# Autodesk Inventor assembly: Assembly3
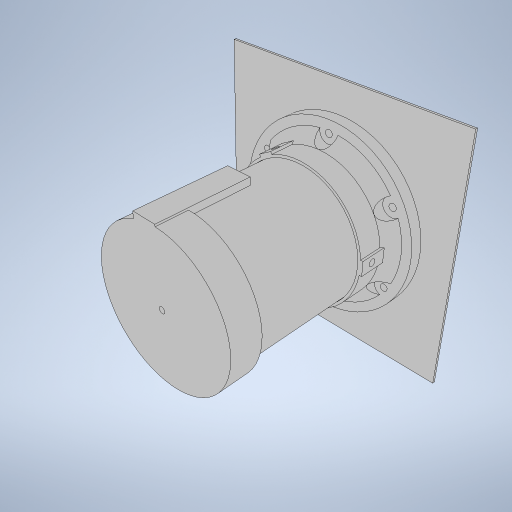
[picture p0: Inventor's stored thumbnail of the model, 512x512]
Saved by Autodesk Inventor 2023 (Build 270158000, 158)
## iProperties
Created: 2023-04-27
Part Number: Assembly3
Document SubType Name: Assembly
Designer: alexa
Author: alexa
## Documents named in this file (5)
- D:\Projects\Mushroom\Assembly3.iam
- D:\Projects\Mushroom\uppe sheet.ipt
- D:\Projects\Mushroom\holding ring.ipt
- D:\Projects\Mushroom\Pipe.ipt
- D:\Projects\Mushroom\Disc.ipt
## Components (4 placed, 4 different names)
1. uppe sheet:1 — Mate:1, Insert:1, Insert:2
2. holding ring:1 — Mate:1, Insert:1
3. Pipe:1 — Insert:2, Insert:3
4. Disc:1 — Insert:3
## Relationships (4: Insert 3, Mate 1)
- Mate:1: uppe sheet:1 ↔ holding ring:1
- Insert:1: uppe sheet:1 ↔ holding ring:1
- Insert:2: uppe sheet:1 ↔ Pipe:1
- Insert:3 (5 mm): Pipe:1 ↔ Disc:1
